# Autodesk Inventor assembly: 446 Module
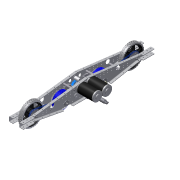
[picture p0: Inventor's stored thumbnail of the model, 180x180]
Saved by Autodesk Inventor 2013 (Build 170138000, 138)
## iProperties
Created: 2012-10-14
Part Number: 446 Module
Document SubType Name: Assembly
Designer: Nemo
Mass: 7075.66 g
Surface Area: 10398.9 cm^2
Volume: 2402.45 cm^3
Density: 2.94519 g/cm^3
Author: Nemo
## Documents named in this file (11)
- H:\Nemo\Documents\Robotics\COTS Parts\Gearboxes\446 Module.iam
- H:\Nemo\Documents\Robotics\COTS Parts\Gearboxes\Housings\446 Drive Plate v4.ipt
- H:\Nemo\Documents\Robotics\COTS Parts\Gearboxes\Shafts\446 Cluster Shaft subassembly.iam
- H:\Nemo\Documents\Robotics\COTS Parts\Gearboxes\Shafts\446 Shifter Shaft.iam
- H:\Nemo\Documents\Robotics\COTS Parts\Gearboxes\Shafts\446 idler shaft.iam
- H:\Nemo\Documents\Robotics\COTS Parts\Gearboxes\Shafts\446 Wheel Shaft.iam
- H:\Nemo\Documents\Robotics\COTS Parts\Gearboxes\Shafts\446 FIRST HiGrip Wheel Shaft.iam
- H:\Nemo\Documents\Robotics\COTS Parts\Gearboxes\Shifters\Shifter Cylinder Subassembly.iam
- H:\Nemo\Documents\Robotics\COTS Parts\Motors\CIM motor 12T for 446.iam
- H:\Nemo\Documents\Robotics\COTS Parts\Gearboxes\Housings\446 Structural Spacer.iam
- H:\Nemo\Documents\Robotics\COTS Parts\Gearboxes\Shafts\446 Roller Chain.ipt
## Components (19 placed, 10 different names)
1. 446 Drive Plate v4:1 — Flush:1, Mate:1, Mate:2, Mate:3, Flush:4, Flush:5, Insert:1, Insert:2, Insert:3, Insert:4, Insert:5, Insert:6, Insert:7, Insert:8, Insert:11, Insert:12, Insert:13, Insert:14
2. 446 Drive Plate v4:2 — Mate:3, Flush:4, Flush:5, Mate:4, Mate:5, Mate:6, Insert:9, Mate:7, Insert:10, Mate:8
3. 446 Cluster Shaft subassembly:1 [sub-assembly] — Insert:1
4. 446 Shifter Shaft:1 [sub-assembly] — Insert:2
5. 446 idler shaft:1 [sub-assembly] — Insert:4
6. 446 idler shaft:2 [sub-assembly] — Insert:3
7. 446 Wheel Shaft:1 [sub-assembly] — Insert:6, Flush:6, Mate:9, Mate:10
8. 446 Wheel Shaft:2 [sub-assembly] — Insert:5, Flush:7, Mate:11, Mate:12
9. 446 FIRST HiGrip Wheel Shaft:1 [sub-assembly] — Insert:8, Flush:6
10. 446 FIRST HiGrip Wheel Shaft:2 [sub-assembly] — Insert:7, Flush:7
11. Shifter Cylinder Subassembly:1 [sub-assembly] — Mate:4, Mate:5, Mate:6
12. CIM motor 12T for 446:1 [sub-assembly] — Insert:9, Mate:7
13. CIM motor 12T for 446:2 [sub-assembly] — Insert:10, Mate:8
14. 446 Structural Spacer:1 [sub-assembly] — Insert:13
15. 446 Structural Spacer:2 [sub-assembly] — Insert:14
16. 446 Structural Spacer:3 [sub-assembly] — Insert:12
17. 446 Structural Spacer:4 [sub-assembly] — Insert:11
18. Roller Chain:1 — Mate:11, Mate:12
19. Roller Chain:2 — Mate:9, Mate:10
## Relationships (31: Insert 14, Mate 12, Flush 5)
- Flush:1: 446 Drive Plate v4:1
- Mate:1: 446 Drive Plate v4:1
- Mate:2: 446 Drive Plate v4:1
- Mate:3 (66.04 mm): 446 Drive Plate v4:1 ↔ 446 Drive Plate v4:2
- Flush:4: 446 Drive Plate v4:1 ↔ 446 Drive Plate v4:2
- Flush:5: 446 Drive Plate v4:1 ↔ 446 Drive Plate v4:2
- Insert:1: 446 Drive Plate v4:1 ↔ 446 Cluster Shaft subassembly:1
- Insert:2: 446 Drive Plate v4:1 ↔ 446 Shifter Shaft:1
- Insert:3: 446 Drive Plate v4:1 ↔ 446 idler shaft:2
- Insert:4: 446 Drive Plate v4:1 ↔ 446 idler shaft:1
- Insert:5: 446 Drive Plate v4:1 ↔ 446 Wheel Shaft:2
- Insert:6: 446 Drive Plate v4:1 ↔ 446 Wheel Shaft:1
- Insert:7: 446 Drive Plate v4:1 ↔ 446 FIRST HiGrip Wheel Shaft:2
- Insert:8: 446 Drive Plate v4:1 ↔ 446 FIRST HiGrip Wheel Shaft:1
- Flush:6: 446 Wheel Shaft:1 ↔ 446 FIRST HiGrip Wheel Shaft:1
- Flush:7: 446 Wheel Shaft:2 ↔ 446 FIRST HiGrip Wheel Shaft:2
- Mate:4: 446 Drive Plate v4:2 ↔ Shifter Cylinder Subassembly:1
- Mate:5: 446 Drive Plate v4:2 ↔ Shifter Cylinder Subassembly:1
- Mate:6: 446 Drive Plate v4:2 ↔ Shifter Cylinder Subassembly:1
- Insert:9: 446 Drive Plate v4:2 ↔ CIM motor 12T for 446:1
- Mate:7: 446 Drive Plate v4:2 ↔ CIM motor 12T for 446:1
- Insert:10: 446 Drive Plate v4:2 ↔ CIM motor 12T for 446:2
- Mate:8: 446 Drive Plate v4:2 ↔ CIM motor 12T for 446:2
- Insert:11: 446 Drive Plate v4:1 ↔ 446 Structural Spacer:4
- Insert:12: 446 Drive Plate v4:1 ↔ 446 Structural Spacer:3
- Insert:13: 446 Drive Plate v4:1 ↔ 446 Structural Spacer:1
- Insert:14: 446 Drive Plate v4:1 ↔ 446 Structural Spacer:2
- Mate:9: 446 Wheel Shaft:1 ↔ Roller Chain:2
- Mate:10: 446 Wheel Shaft:1 ↔ Roller Chain:2
- Mate:11: 446 Wheel Shaft:2 ↔ Roller Chain:1
- Mate:12: 446 Wheel Shaft:2 ↔ Roller Chain:1
